# Autodesk Inventor assembly: Cover V3 Assembly
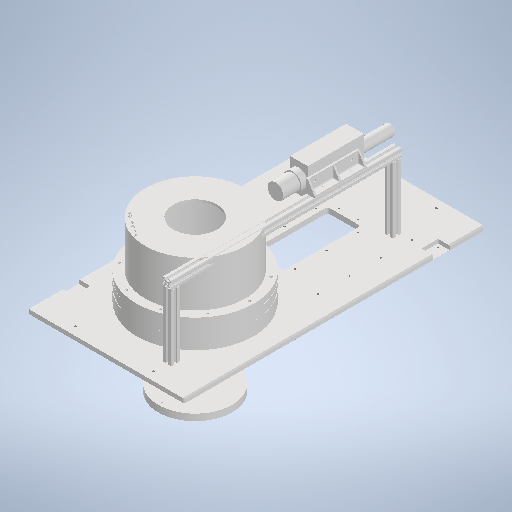
[picture p0: Inventor's stored thumbnail of the model, 512x512]
Saved by Autodesk Inventor 2025.2 (Build 292293000, 293)
## iProperties
Created: 2025-06-17
Part Number: Cover V3 Assembly
Document SubType Name: Assembly
Designer: mumin
Author: mumin
## Documents named in this file (10)
- C:\GitHub\In-situ-monitoring-of-powder-bed-fusion-additive-manufacturing\system_development\Orichalcum\v0.3\Cover v3 Assembly\Cover V3 Assembly.iam
- C:\GitHub\In-situ-monitoring-of-powder-bed-fusion-additive-manufacturing\system_development\Orichalcum\v0.3\Cover v3 Assembly\2020 Legs (150mm).ipt
- C:\GitHub\In-situ-monitoring-of-powder-bed-fusion-additive-manufacturing\system_development\Orichalcum\v0.3\Cover v3 Assembly\2020 LV-GVS Beam (530).ipt
- C:\GitHub\In-situ-monitoring-of-powder-bed-fusion-additive-manufacturing\system_development\Orichalcum\v0.3\Cover v3 Assembly\LV_Bracket_2.ipt
- C:\GitHub\In-situ-monitoring-of-powder-bed-fusion-additive-manufacturing\system_development\Orichalcum\v0.3\Cover v3 Assembly\12mm Cover.ipt
- C:\GitHub\In-situ-monitoring-of-powder-bed-fusion-additive-manufacturing\system_development\Orichalcum\v0.3\Cover v3 Assembly\Lower Ring (30mm).ipt
- C:\GitHub\In-situ-monitoring-of-powder-bed-fusion-additive-manufacturing\system_development\Orichalcum\v0.3\Cover v3 Assembly\Build Plate.ipt
- C:\GitHub\In-situ-monitoring-of-powder-bed-fusion-additive-manufacturing\system_development\Orichalcum\v0.3\Cover v3 Assembly\Middle Ring (20mm).ipt
- C:\GitHub\In-situ-monitoring-of-powder-bed-fusion-additive-manufacturing\system_development\Orichalcum\v0.3\Cover v3 Assembly\Cylinder Housing.ipt
- C:\GitHub\In-situ-monitoring-of-powder-bed-fusion-additive-manufacturing\system_development\Orichalcum\v0.3\Cover v3 Assembly\Updated Laser Scanner.ipt
## Components (10 placed, 9 different names)
1. 2020 Legs (150mm):1 — Flush:1, Flush:2, Mate:1, Insert:1
2. 2020 Legs (150mm):2 — Mate:2, Flush:3, Flush:4
3. 2020 LV-GVS Beam (530):1 — Flush:1, Flush:2, Mate:1, Mate:2, Flush:3, Flush:4, Mate:3, Flush:5
4. LV_Bracket_2:1 — Mate:3, Flush:5, Insert:9
5. 12mm Cover:1 — Insert:1, Insert:2, Insert:3, Insert:4
6. Lower Ring (30mm):1 — Insert:2, Insert:3, Insert:5, Insert:6
7. Build Plate:1 — Insert:4
8. Middle Ring (20mm):1 — Insert:5, Insert:6, Insert:7, Insert:8
9. Cylinder Housing:1 — Insert:7, Insert:8
10. Updated Laser Scanner:1 — Insert:9
## Relationships (17: Insert 9, Flush 5, Mate 3)
- Flush:1: 2020 Legs (150mm):1 ↔ 2020 LV-GVS Beam (530):1
- Flush:2: 2020 Legs (150mm):1 ↔ 2020 LV-GVS Beam (530):1
- Mate:1: 2020 Legs (150mm):1 ↔ 2020 LV-GVS Beam (530):1
- Mate:2: 2020 Legs (150mm):2 ↔ 2020 LV-GVS Beam (530):1
- Flush:3: 2020 Legs (150mm):2 ↔ 2020 LV-GVS Beam (530):1
- Flush:4: 2020 Legs (150mm):2 ↔ 2020 LV-GVS Beam (530):1
- Mate:3: 2020 LV-GVS Beam (530):1 ↔ LV_Bracket_2:1
- Flush:5: 2020 LV-GVS Beam (530):1 ↔ LV_Bracket_2:1
- Insert:1: 2020 Legs (150mm):1 ↔ 12mm Cover:1
- Insert:2: 12mm Cover:1 ↔ Lower Ring (30mm):1
- Insert:3: 12mm Cover:1 ↔ Lower Ring (30mm):1
- Insert:4 (150 mm): 12mm Cover:1 ↔ Build Plate:1
- Insert:5: Lower Ring (30mm):1 ↔ Middle Ring (20mm):1
- Insert:6: Lower Ring (30mm):1 ↔ Middle Ring (20mm):1
- Insert:7: Middle Ring (20mm):1 ↔ Cylinder Housing:1
- Insert:8: Middle Ring (20mm):1 ↔ Cylinder Housing:1
- Insert:9: LV_Bracket_2:1 ↔ Updated Laser Scanner:1
